# Autodesk Inventor assembly: powerDistAssem
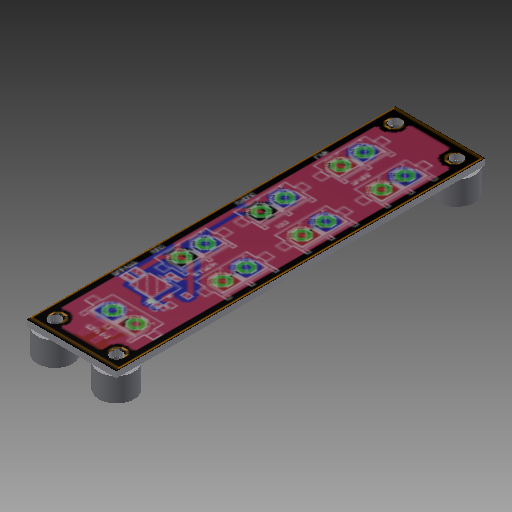
[picture p0: Inventor's stored thumbnail of the model, 512x512]
Saved by Autodesk Inventor 2018 (Build 220112000, 112)
## iProperties
Created: 2018-08-04
Part Number: powerDistAssem
Document SubType Name: Assembly
Designer: Cole Tucker
Mass: 5.60956 g
Surface Area: 66.9552 cm^2
Volume: 5.38311 cm^3
Density: 1.04207 g/cm^3
Author: Cole Tucker
## Documents named in this file (3)
- C:\Users\Cole Tucker\OneDrive\FRC-mxpProject\Cad\ControlCase\Inventor\powerDistAssem.iam
- C:\Users\Cole Tucker\OneDrive\FRC-mxpProject\Cad\ControlCase\Inventor\powerDist.ipt
- C:\Users\Cole Tucker\OneDrive\FRC-mxpProject\Cad\ControlCase\Inventor\powerDistSpacer.ipt
## Components (5 placed, 2 different names)
1. powerDist:1 — Mate:1, Mate:2, Mate:3, Mate:4, Mate:5, Mate:6, Mate:7, Mate:8
2. powerDistSpacer:1 — Mate:3, Mate:6
3. powerDistSpacer:2 — Mate:1, Mate:7
4. powerDistSpacer:3 — Mate:2, Mate:8
5. powerDistSpacer:4 — Mate:4, Mate:5
## Relationships (8: Mate 8)
- Mate:1: powerDist:1 ↔ powerDistSpacer:2
- Mate:2: powerDist:1 ↔ powerDistSpacer:3
- Mate:3: powerDist:1 ↔ powerDistSpacer:1
- Mate:4: powerDist:1 ↔ powerDistSpacer:4
- Mate:5: powerDist:1 ↔ powerDistSpacer:4
- Mate:6: powerDist:1 ↔ powerDistSpacer:1
- Mate:7: powerDist:1 ↔ powerDistSpacer:2
- Mate:8: powerDist:1 ↔ powerDistSpacer:3
